# Autodesk Inventor assembly: Pancake_Timing Assy 2_3 Lanes
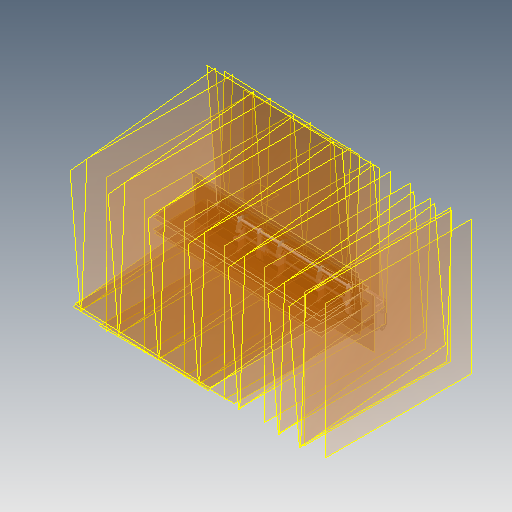
[picture p0: Inventor's stored thumbnail of the model, 512x512]
Saved by Autodesk Inventor 2018.1 (Build 221171000, 171)
## iProperties
Created: 2019-02-11
Part Number: Pancake_Timing Assy 2_3 Lanes
Document SubType Name: Assembly
Designer: James
Author: James
## Documents named in this file (11)
- C:\Users\admin\Desktop\Ball-Machine\Pancake Sort\Pancake - 3 Lanes\Pancake_Timing Assy 2_3 Lanes.iam
- C:\Users\admin\Desktop\Ball-Machine\Prototype CAD\Selection Sort - 40mm\Nyloc Nut - M4.ipt
- C:\Users\admin\Desktop\Ball-Machine\Prototype CAD\Selection Sort - 40mm\Socket Csk Screw - (A2) - M4 x  16.ipt
- C:\Users\admin\Desktop\Ball-Machine\Prototype CAD\Selection Sort - 40mm\Socket Cap Screw - Standard - (A2) - M4 x 16.ipt
- C:\Users\admin\Desktop\Ball-Machine\Pancake Sort\Pancake_Angle Bracket.ipt
- C:\Users\admin\Desktop\Ball-Machine\Pancake Sort\Pancake_PVC Pipe 2.ipt
- C:\Users\admin\Desktop\Ball-Machine\Pancake Sort\Pancake_Bracket.ipt
- C:\Users\admin\Desktop\Ball-Machine\Pancake Sort\Pancake - 3 Lanes\Pancake_Timing Backboard 2_3 Lanes.ipt
- C:\Users\admin\Desktop\Ball-Machine\Pancake Sort\Pancake - 3 Lanes\Pancake_Timing Assy_Lever Shaft 2_3 Lanes.iam
- C:\Users\admin\Desktop\Ball-Machine\Pancake Sort\Pancake - 3 Lanes\Pancake_Timing Assy_Star Shaft 2_3 Lanes.iam
- C:\Users\admin\Desktop\Ball-Machine\Pancake Sort\FWSRS-D12-V4.5-E2.5-T3_.ipt
## Components (48 placed, 10 different names)
1. Pancake_Timing Backboard 2_3 Lanes:1 — Angle:2, Tangent:1, Mate:93, Mate:94, Mate:95, Mate:96, Flush:34, Mate:104, Mate:105, Mate:106, Flush:36, Mate:107, Mate:108, Mate:115, Flush:37, Mate:116, Mate:117, Mate:118, Mate:119, Mate:134, Mate:135, Mate:136, Mate:137, Mate:138, Mate:139, Mate:158, Mate:159, Mate:163, Mate:164
2. Pancake_Timing Assy_Lever Shaft 2_3 Lanes:1 [sub-assembly] — Mate:140, Mate:141, Mate:142, Mate:143
3. Pancake_Timing Assy_Star Shaft 2_3 Lanes:1 [sub-assembly] — Angle:2, Mate:144, Mate:145, Mate:148, Mate:149, Mate:150
4. Pancake_Angle Bracket:3 — Mate:104, Mate:105, Mate:106, Flush:36, Mate:124, Mate:125, Mate:126, Mate:127
5. Pancake_Angle Bracket:4 — Mate:115, Flush:37, Mate:118, Mate:119, Mate:131, Mate:167, Mate:168, Mate:169
6. Socket Cap Screw - Standard - (A2) - M4 x 16:10
7. Socket Cap Screw - Standard - (A2) - M4 x 16:7
8. Socket Cap Screw - Standard - (A2) - M4 x 16:8
9. Nyloc Nut - M4:17 — Mate:108
10. Nyloc Nut - M4:18 — Mate:107
11. Nyloc Nut - M4:27 — Mate:117
12. Socket Cap Screw - Standard - (A2) - M4 x 16:9
13. Nyloc Nut - M4:28 — Mate:116
14. Socket Cap Screw - Standard - (A2) - M4 x 16:11 — Flush:98, Mate:125, Mate:126
15. Nyloc Nut - M4:37 — Flush:99, Mate:127
16. Socket Cap Screw - Standard - (A2) - M4 x 16:12 — Flush:98, Mate:124
17. Nyloc Nut - M4:38 — Flush:99
18. Nyloc Nut - M4:39 — Flush:101, Mate:131, Mate:171
19. Nyloc Nut - M4:40 — Flush:101, Mate:170
20. Pancake_Bracket:1 — Mate:134, Mate:136, Mate:137, Mate:140, Mate:144, Mate:149, Mate:150, Mate:160, Mate:161, Mate:162
21. Pancake_Bracket:2 — Mate:135, Mate:138, Mate:139, Mate:141, Mate:142, Mate:143, Mate:145, Mate:148, Mate:155, Mate:156, Mate:157
22. Socket Cap Screw - Standard - (A2) - M4 x 16:15 — Flush:104, Mate:160, Mate:161
23. Nyloc Nut - M4:41 — Mate:164
24. Socket Cap Screw - Standard - (A2) - M4 x 16:16 — Flush:104, Mate:162
25. Nyloc Nut - M4:42 — Mate:163
26. Socket Cap Screw - Standard - (A2) - M4 x 16:17 — Flush:105, Mate:157
27. Nyloc Nut - M4:43 — Mate:159
28. Socket Cap Screw - Standard - (A2) - M4 x 16:18 — Flush:105, Mate:155, Mate:156
29. Nyloc Nut - M4:44 — Mate:158
30. Socket Csk Screw - (A2) - M4 x  16:9 — Mate:168, Mate:171
31. FWSRS-D12-V4.5-E2.5-T3.0:1 — Flush:106, Mate:167
32. Socket Csk Screw - (A2) - M4 x  16:10 — Mate:169, Mate:170
33. FWSRS-D12-V4.5-E2.5-T3.0:2 — Flush:106
34. Pancake_PVC Pipe 2:1 — Angle:1, Mate:54, Tangent:1, Mate:93, Mate:94, Mate:97, Flush:102
35. Socket Csk Screw - (A2) - M4 x  16:1 — Mate:54, Flush:21, Mate:57, Flush:34
36. Socket Csk Screw - (A2) - M4 x  16:2 — Flush:21, Mate:58, Mate:97
37. Nyloc Nut - M4:1 — Mate:58, Mate:95
38. Nyloc Nut - M4:2 — Mate:57, Mate:96
39. Pancake_PVC Pipe 2:2
40. Socket Csk Screw - (A2) - M4 x  16:3
41. Socket Csk Screw - (A2) - M4 x  16:4
42. Nyloc Nut - M4:29
43. Nyloc Nut - M4:30
44. Pancake_PVC Pipe 2:3
45. Socket Csk Screw - (A2) - M4 x  16:5
46. Socket Csk Screw - (A2) - M4 x  16:6
47. Nyloc Nut - M4:31
48. Nyloc Nut - M4:32
## Component patterns: (3 elements, first: Pancake_PVC Pipe 2:1 + Socket Csk Screw - (A2) - M4 x  16:1 + Socket Csk Screw - (A2) - M4 x  16:2 + Nyloc Nut - M4:1 + Nyloc Nut - M4:2)
## Relationships (94: Mate 73, Flush 16, Tangent 3, Angle 2)
- Angle:1 (0 deg): Pancake_PVC Pipe 2:1
- Flush:11 (62.5 mm)
- [Flush]: Pancake_Timing Backboard 2_3 Lanes:1
- [Flush]: Pancake_Timing Backboard 2_3 Lanes:1
- [Flush]: Pancake_Timing Backboard 2_3 Lanes:1
- Mate:54: Pancake_PVC Pipe 2:1 ↔ Socket Csk Screw - (A2) - M4 x  16:1
- Flush:21: Socket Csk Screw - (A2) - M4 x  16:1 ↔ Socket Csk Screw - (A2) - M4 x  16:2
- Mate:57: Socket Csk Screw - (A2) - M4 x  16:1 ↔ Nyloc Nut - M4:2
- Mate:58: Socket Csk Screw - (A2) - M4 x  16:2 ↔ Nyloc Nut - M4:1
- Angle:2 (0 deg): Pancake_Timing Backboard 2_3 Lanes:1 ↔ Pancake_Timing Assy_Star Shaft 2_3 Lanes:1
- Tangent:1: Pancake_Timing Backboard 2_3 Lanes:1 ↔ Pancake_PVC Pipe 2:1
- Mate:93: Pancake_Timing Backboard 2_3 Lanes:1 ↔ Pancake_PVC Pipe 2:1
- Mate:94: Pancake_Timing Backboard 2_3 Lanes:1 ↔ Pancake_PVC Pipe 2:1
- Mate:95: Pancake_Timing Backboard 2_3 Lanes:1 ↔ Nyloc Nut - M4:1
- Mate:96: Pancake_Timing Backboard 2_3 Lanes:1 ↔ Nyloc Nut - M4:2
- Flush:34 (-5 mm): Pancake_Timing Backboard 2_3 Lanes:1 ↔ Socket Csk Screw - (A2) - M4 x  16:1
- Mate:97: Pancake_PVC Pipe 2:1 ↔ Socket Csk Screw - (A2) - M4 x  16:2
- [Mate]: Pancake_Angle Bracket:3 ↔ Socket Cap Screw - Standard - (A2) - M4 x 16:8
- [Mate]: Pancake_Angle Bracket:3 ↔ Socket Cap Screw - Standard - (A2) - M4 x 16:8
- [Mate]: Pancake_Angle Bracket:3 ↔ Socket Cap Screw - Standard - (A2) - M4 x 16:7
- [Mate]: Pancake_Angle Bracket:3 ↔ Socket Cap Screw - Standard - (A2) - M4 x 16:7
- [Mate]: Socket Cap Screw - Standard - (A2) - M4 x 16:8 ↔ Nyloc Nut - M4:18
- [Mate]: Socket Cap Screw - Standard - (A2) - M4 x 16:7 ↔ Nyloc Nut - M4:17
- Mate:104: Pancake_Timing Backboard 2_3 Lanes:1 ↔ Pancake_Angle Bracket:3
- Mate:105: Pancake_Timing Backboard 2_3 Lanes:1 ↔ Pancake_Angle Bracket:3
- Mate:106: Pancake_Timing Backboard 2_3 Lanes:1 ↔ Pancake_Angle Bracket:3
- Flush:36: Pancake_Timing Backboard 2_3 Lanes:1 ↔ Pancake_Angle Bracket:3
- Mate:107: Pancake_Timing Backboard 2_3 Lanes:1 ↔ Nyloc Nut - M4:18
- Mate:108: Pancake_Timing Backboard 2_3 Lanes:1 ↔ Nyloc Nut - M4:17
- [Mate]: Pancake_Angle Bracket:4 ↔ Socket Cap Screw - Standard - (A2) - M4 x 16:10
- [Mate]: Pancake_Angle Bracket:4 ↔ Socket Cap Screw - Standard - (A2) - M4 x 16:10
- [Mate]: Pancake_Angle Bracket:4 ↔ Socket Cap Screw - Standard - (A2) - M4 x 16:9
- [Mate]: Pancake_Angle Bracket:4 ↔ Socket Cap Screw - Standard - (A2) - M4 x 16:9
- [Mate]: Socket Cap Screw - Standard - (A2) - M4 x 16:10 ↔ Nyloc Nut - M4:27
- [Mate]: Socket Cap Screw - Standard - (A2) - M4 x 16:9 ↔ Nyloc Nut - M4:28
- Mate:115: Pancake_Timing Backboard 2_3 Lanes:1 ↔ Pancake_Angle Bracket:4
- Flush:37: Pancake_Timing Backboard 2_3 Lanes:1 ↔ Pancake_Angle Bracket:4
- Mate:116: Pancake_Timing Backboard 2_3 Lanes:1 ↔ Nyloc Nut - M4:28
- Mate:117: Pancake_Timing Backboard 2_3 Lanes:1 ↔ Nyloc Nut - M4:27
- Mate:118: Pancake_Timing Backboard 2_3 Lanes:1 ↔ Pancake_Angle Bracket:4
- Mate:119: Pancake_Timing Backboard 2_3 Lanes:1 ↔ Pancake_Angle Bracket:4
- [Mate]: Socket Cap Screw - Standard - (A2) - M4 x 16:11 ↔ Nyloc Nut - M4:37
- [Mate]: Socket Cap Screw - Standard - (A2) - M4 x 16:12 ↔ Nyloc Nut - M4:38
- Flush:98: Socket Cap Screw - Standard - (A2) - M4 x 16:11 ↔ Socket Cap Screw - Standard - (A2) - M4 x 16:12
- Mate:124: Pancake_Angle Bracket:3 ↔ Socket Cap Screw - Standard - (A2) - M4 x 16:12
- Mate:125: Pancake_Angle Bracket:3 ↔ Socket Cap Screw - Standard - (A2) - M4 x 16:11
- Mate:126 (5 mm): Pancake_Angle Bracket:3 ↔ Socket Cap Screw - Standard - (A2) - M4 x 16:11
- Flush:99: Nyloc Nut - M4:37 ↔ Nyloc Nut - M4:38
- Mate:127: Pancake_Angle Bracket:3 ↔ Nyloc Nut - M4:37
- Flush:101: Nyloc Nut - M4:39 ↔ Nyloc Nut - M4:40
- Mate:131: Pancake_Angle Bracket:4 ↔ Nyloc Nut - M4:39
- Flush:102 (65 mm): Pancake_PVC Pipe 2:1
- Flush:103 (35 mm)
- Mate:134: Pancake_Timing Backboard 2_3 Lanes:1 ↔ Pancake_Bracket:1
- Mate:135: Pancake_Timing Backboard 2_3 Lanes:1 ↔ Pancake_Bracket:2
- Mate:136: Pancake_Timing Backboard 2_3 Lanes:1 ↔ Pancake_Bracket:1
- Mate:137: Pancake_Timing Backboard 2_3 Lanes:1 ↔ Pancake_Bracket:1
- Mate:138: Pancake_Timing Backboard 2_3 Lanes:1 ↔ Pancake_Bracket:2
- Mate:139: Pancake_Timing Backboard 2_3 Lanes:1 ↔ Pancake_Bracket:2
- Mate:140: Pancake_Timing Assy_Lever Shaft 2_3 Lanes:1 ↔ Pancake_Bracket:1
- Mate:141: Pancake_Timing Assy_Lever Shaft 2_3 Lanes:1 ↔ Pancake_Bracket:2
- Mate:142: Pancake_Timing Assy_Lever Shaft 2_3 Lanes:1 ↔ Pancake_Bracket:2
- Mate:143: Pancake_Timing Assy_Lever Shaft 2_3 Lanes:1 ↔ Pancake_Bracket:2
- Mate:144: Pancake_Timing Assy_Star Shaft 2_3 Lanes:1 ↔ Pancake_Bracket:1
- Mate:145: Pancake_Timing Assy_Star Shaft 2_3 Lanes:1 ↔ Pancake_Bracket:2
- Mate:148: Pancake_Timing Assy_Star Shaft 2_3 Lanes:1 ↔ Pancake_Bracket:2
- Mate:149: Pancake_Timing Assy_Star Shaft 2_3 Lanes:1 ↔ Pancake_Bracket:1
- Mate:150: Pancake_Timing Assy_Star Shaft 2_3 Lanes:1 ↔ Pancake_Bracket:1
- [Mate]: Socket Cap Screw - Standard - (A2) - M4 x 16:15 ↔ Nyloc Nut - M4:41
- [Mate]: Socket Cap Screw - Standard - (A2) - M4 x 16:16 ↔ Nyloc Nut - M4:42
- [Mate]: Socket Cap Screw - Standard - (A2) - M4 x 16:17 ↔ Nyloc Nut - M4:43
- [Mate]: Socket Cap Screw - Standard - (A2) - M4 x 16:18 ↔ Nyloc Nut - M4:44
- Flush:104: Socket Cap Screw - Standard - (A2) - M4 x 16:15 ↔ Socket Cap Screw - Standard - (A2) - M4 x 16:16
- Flush:105: Socket Cap Screw - Standard - (A2) - M4 x 16:17 ↔ Socket Cap Screw - Standard - (A2) - M4 x 16:18
- Mate:155: Pancake_Bracket:2 ↔ Socket Cap Screw - Standard - (A2) - M4 x 16:18
- Mate:156: Pancake_Bracket:2 ↔ Socket Cap Screw - Standard - (A2) - M4 x 16:18
- Mate:157: Pancake_Bracket:2 ↔ Socket Cap Screw - Standard - (A2) - M4 x 16:17
- Mate:158: Pancake_Timing Backboard 2_3 Lanes:1 ↔ Nyloc Nut - M4:44
- Mate:159: Pancake_Timing Backboard 2_3 Lanes:1 ↔ Nyloc Nut - M4:43
- Mate:160: Pancake_Bracket:1 ↔ Socket Cap Screw - Standard - (A2) - M4 x 16:15
- Mate:161: Pancake_Bracket:1 ↔ Socket Cap Screw - Standard - (A2) - M4 x 16:15
- Mate:162: Pancake_Bracket:1 ↔ Socket Cap Screw - Standard - (A2) - M4 x 16:16
- Mate:163: Pancake_Timing Backboard 2_3 Lanes:1 ↔ Nyloc Nut - M4:42
- Mate:164: Pancake_Timing Backboard 2_3 Lanes:1 ↔ Nyloc Nut - M4:41
- [Mate]: Socket Csk Screw - (A2) - M4 x  16:9 ↔ FWSRS-D12-V4.5-E2.5-T3.0:1
- [Tangent]: Socket Csk Screw - (A2) - M4 x  16:9 ↔ FWSRS-D12-V4.5-E2.5-T3.0:1
- [Mate]: Socket Csk Screw - (A2) - M4 x  16:10 ↔ FWSRS-D12-V4.5-E2.5-T3.0:2
- [Tangent]: Socket Csk Screw - (A2) - M4 x  16:10 ↔ FWSRS-D12-V4.5-E2.5-T3.0:2
- Flush:106: FWSRS-D12-V4.5-E2.5-T3.0:1 ↔ FWSRS-D12-V4.5-E2.5-T3.0:2
- Mate:167 (5 mm): Pancake_Angle Bracket:4 ↔ FWSRS-D12-V4.5-E2.5-T3.0:1
- Mate:168: Pancake_Angle Bracket:4 ↔ Socket Csk Screw - (A2) - M4 x  16:9
- Mate:169: Pancake_Angle Bracket:4 ↔ Socket Csk Screw - (A2) - M4 x  16:10
- Mate:170: Nyloc Nut - M4:40 ↔ Socket Csk Screw - (A2) - M4 x  16:10
- Mate:171: Nyloc Nut - M4:39 ↔ Socket Csk Screw - (A2) - M4 x  16:9
## Named parameters: d168_d139_d131 = 0 mm, d169_d140_d132 = 0 mm, d170_d141_d133 = 0 mm, d171_d142_d134 = 0 mm, d172_d149 = 0 mm, d173_d150 = 0 mm, d185_d131 = 0 mm, d186_d132 = 0 mm, d187_d133 = 0 mm, d188_d134 = 0 mm, d189_d137 = 0 mm, d190_d138 = 0 mm, d211_d172_d149 = 0 mm, d212_d172_d149 = 0 mm, d248_d172_d149 = 0 mm, d249_d172_d149 = 0 mm, d250_d172_d149 = 0 mm, d251_d172_d149 = 0 mm, d266_d387 = 0 mm, d267_d388 = 0 mm
